# Autodesk Inventor assembly: 细轴四方轴套用的螺丝螺帽套
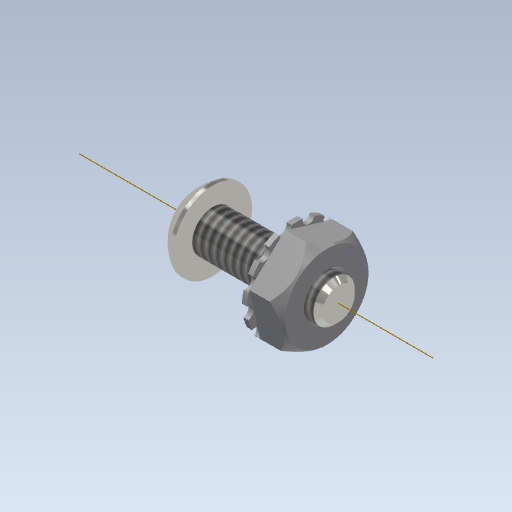
[picture p0: Inventor's stored thumbnail of the model, 512x512]
Saved by Autodesk Inventor 2020 (Build 240168000, 168)
## iProperties
Created: 2019-05-20
Part Number: 细轴四方轴套用的螺丝螺帽套
Material: 常规
Document SubType Name: Assembly
Designer: aresp
Mass: 3.28505 g
Surface Area: 6.70102 cm^2
Volume: 0.424519 cm^3
Density: 7.7383 g/cm^3
Author: aresp
## Documents named in this file (3)
- C:\towerTakeOverCad\ncrCadLib\细轴四方轴套用的螺丝螺帽套.iam
- C:\towerTakeOverCad\ncrCadLib\螺丝螺帽\Screw 8-32 x 0.500'' 三号.ipt
- C:\towerTakeOverCad\ncrCadLib\螺丝螺帽\普通螺帽.ipt
## Components (2 placed, 2 different names)
1. Screw 8-32 x 0.500'' 三号:1 — 配合:2
2. 普通螺帽:1 — 配合:2
## Relationships (2: Mate 2)
- [Mate]: Screw 8-32 x 0.500'' 三号:1 ↔ 普通螺帽:1
- 配合:2 [Mate] (7.925 mm): Screw 8-32 x 0.500'' 三号:1 ↔ 普通螺帽:1
